# Autodesk Inventor assembly: Baugruppe2
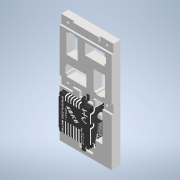
[picture p0: Inventor's stored thumbnail of the model, 180x180]
Saved by Autodesk Inventor 2022 (Build 260153000, 153)
## iProperties
Created: 2022-05-05
Part Number: Baugruppe2
Document SubType Name: Assembly
Designer: 123St
Author: 123St
## Documents named in this file (3)
- D:\Eigene Dateien\Desktop\UNI\Semester 5\Praktikum\DaVinci\Ueberarbeiteter DaVincikopf\Baugruppe2.iam
- D:\Eigene Dateien\Desktop\UNI\Semester 5\Praktikum\DaVinci\Ueberarbeiteter DaVincikopf\Fuehrungsgrundplatte_V3.ipt
- D:\Eigene Dateien\Desktop\UNI\Semester 5\Praktikum\DaVinci\Ueberarbeiteter DaVincikopf\JX BLS-HV7146MG.iam
## Components (2 placed, 2 different names)
1. Fuehrungsgrundplatte_V3:1 — Fluchtend:1, Passend:1, Passend:2
2. JX BLS-HV7146MG:1 [sub-assembly] — Fluchtend:1, Passend:1, Passend:2
## Relationships (3: Mate 2, Flush 1)
- Fluchtend:1 [Flush] (-5 mm): Fuehrungsgrundplatte_V3:1 ↔ JX BLS-HV7146MG:1
- Passend:1 [Mate]: Fuehrungsgrundplatte_V3:1 ↔ JX BLS-HV7146MG:1
- Passend:2 [Mate]: Fuehrungsgrundplatte_V3:1 ↔ JX BLS-HV7146MG:1
